# Autodesk Inventor assembly: sb
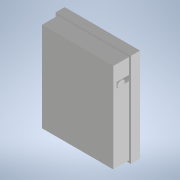
[picture p0: Inventor's stored thumbnail of the model, 180x180]
Saved by Autodesk Inventor 2022 (Build 260153000, 153)
## iProperties
Created: 2025-06-23
Part Number: sb
Document SubType Name: Assembly
Designer: korsh524
Author: korsh524
## Documents named in this file (4)
- C:\git\Olymp20205Smena\Dezign\Stemborad\sb.iam
- C:\git\Olymp20205Smena\Dezign\Stemborad\Stemboard.ipt
- C:\git\Olymp20205Smena\Dezign\Stemborad\btn.ipt
- C:\git\izhplaneta5\speedmetr\models\krishka.ipt
## Components (3 placed, 3 different names)
1. Stemboard:1 — Заподлицо:1
2. btn:1 — Заподлицо:1, Заподлицо:2
3. krishka:1 — Заподлицо:2
## Relationships (2: Flush 2)
- Заподлицо:1 [Flush]: Stemboard:1 ↔ btn:1
- Заподлицо:2 [Flush]: btn:1 ↔ krishka:1
